# Autodesk Inventor assembly: Whole_Assembly
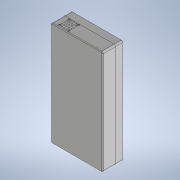
[picture p0: Inventor's stored thumbnail of the model, 180x180]
Saved by Autodesk Inventor 2021 (Build 250183000, 183)
## iProperties
Created: 2020-07-29
Part Number: Whole_Assembly
Document SubType Name: Assembly
Designer: ridvansong
Author: ridvansong
## Documents named in this file (21)
- \\Mac\Home\Documents\OP-1 Project\ipt_files\Whole_Assembly.iam
- \\Mac\Home\Documents\OP-1 Project\ipt_files\Backboard.ipt
- \\Mac\Home\Documents\OP-1 Project\ipt_files\Base.ipt
- \\Mac\Home\Documents\OP-1 Project\ipt_files\Cover.ipt
- \\Mac\Home\Documents\OP-1 Project\ipt_files\RaspPi_Model.ipt
- \\Mac\Home\Documents\OP-1 Project\ipt_files\Fan_Model.ipt
- \\Mac\Home\Documents\OP-1 Project\ipt_files\Battery.ipt
- \\Mac\Home\Documents\OP-1 Project\ipt_files\Battery_Fastener.ipt
- \\Mac\Home\Documents\OP-1 Project\ipt_files\Rotary_Encoder_Model.ipt
- \\Mac\Home\Documents\OP-1 Project\ipt_files\Knob_Base.ipt
- \\Mac\Home\Documents\OP-1 Project\ipt_files\knob.ipt
- \\Mac\Home\Documents\OP-1 Project\ipt_files\Keyboard_Base.ipt
- \\Mac\Home\Documents\OP-1 Project\ipt_files\Small_Button_Base.ipt
- \\Mac\Home\Documents\OP-1 Project\ipt_files\Black_Keyboard_Button_Base.ipt
- \\Mac\Home\Documents\OP-1 Project\ipt_files\Button Prong.ipt
- \\Mac\Home\Documents\OP-1 Project\ipt_files\Black_Keyboard_Button_Prong.ipt
- \\Mac\Home\Documents\OP-1 Project\ipt_files\Keyboard_Prong.ipt
- \\Mac\Home\Documents\OP-1 Project\ipt_files\Small_Button.ipt
- \\Mac\Home\Documents\OP-1 Project\ipt_files\Keyboard Button.ipt
- \\Mac\Home\Documents\OP-1 Project\ipt_files\Black_Keyboard_Button.ipt
- \\Mac\Home\Documents\OP-1 Project\ipt_files\Screen_Model.ipt
## Components (180 placed, 20 different names)
1. Backboard:1 — Mate:1, Mate:3, Mate:4, Mate:15, Mate:16, Mate:17, Mate:18, Angle:1, Angle:2, Angle:3, Angle:4, Mate:25, Mate:35, Mate:37
2. Base:1 — Mate:1, Flush:1, Flush:2, Mate:2, Mate:3, Mate:4, Mate:5, Mate:6, Mate:7, Mate:8, Mate:9, Mate:10, Mate:11, Mate:12, Mate:13, Tangent:1, Tangent:2, Flush:4, Flush:5, Flush:6, Flush:7
3. Cover:1 — Flush:1, Flush:2, Mate:2, Mate:19, Mate:20, Mate:34, Flush:139
4. RaspPi_Model:1 — Mate:8, Mate:9, Mate:10
5. Fan_Model:1 — Mate:5, Mate:6, Mate:7
6. Fan_Model:2 — Mate:11, Mate:12, Mate:13
7. Battery:1 — Tangent:1, Tangent:2, Flush:3
8. Battery_Fastener:1 — Flush:5, Flush:6, Flush:7
9. Rotary_Encoder_Model:1 — Mate:18, Mate:21, Angle:4, Mate:32
10. Rotary_Encoder_Model:2 — Mate:17, Mate:22, Angle:3, Mate:30
11. Rotary_Encoder_Model:3 — Mate:16, Mate:23, Angle:2, Mate:28
12. Rotary_Encoder_Model:4 — Mate:15, Mate:24, Angle:1, Mate:26
13. Knob_Base:1 — Mate:19, Mate:20, Mate:21, Mate:22, Mate:23, Mate:24, Mate:25, Mate:27, Mate:29, Mate:31, Mate:33, Mate:53
14. knob:1 — Mate:26, Mate:27
15. knob:2 — Mate:28, Mate:29
16. knob:3 — Mate:30, Mate:31
17. knob:4 — Mate:32, Mate:33
18. Small_Button_Base:67 — Flush:48, Mate:54, Mate:55, Flush:50, Flush:62, Flush:63, Mate:68, Flush:132, Flush:134
19. Small_Button_Base:68 — Flush:49, Flush:50, Mate:56, Flush:74, Flush:75, Mate:69, Flush:136, Flush:138
20. Black_Keyboard_Button_Base:1 — Flush:53, Flush:54, Flush:55, Flush:56, Flush:57, Mate:64, Mate:65, Flush:107, Flush:108
21. Black_Keyboard_Button_Base:2 — Flush:56, Flush:57, Flush:58, Flush:59, Flush:60, Flush:120, Flush:121
22. Black_Keyboard_Button_Base:3 — Flush:59, Flush:60, Flush:61, Flush:110, Flush:111
23. Black_Keyboard_Button_Base:4 — Flush:62, Flush:63, Flush:64, Flush:65, Flush:66, Mate:66, Flush:123, Flush:124
24. Black_Keyboard_Button_Base:5 — Flush:65, Flush:66, Flush:67, Flush:68, Flush:69, Flush:114, Flush:115
25. Black_Keyboard_Button_Base:6 — Flush:68, Flush:69, Flush:70, Flush:71, Flush:126, Flush:127
26. Black_Keyboard_Button_Base:7 — Flush:71, Flush:72, Flush:74, Flush:117, Flush:118
27. Black_Keyboard_Button_Base:8 — Flush:73, Flush:75, Flush:76, Mate:67, Flush:129, Flush:130
28. Black_Keyboard_Button_Prong:3 — Flush:85, Flush:86, Mate:67
29. Button Prong:31 — Flush:87, Flush:88, Mate:68
30. Button Prong:32 — Flush:89, Flush:90, Mate:69
31. Black_Keyboard_Button:1 — Flush:106, Flush:107, Flush:108, Flush:119
32. Black_Keyboard_Button:2 — Flush:112, Flush:117, Flush:118
33. Black_Keyboard_Button:3 — Flush:109, Flush:110, Flush:111, Flush:122, Flush:131, Flush:133
34. Black_Keyboard_Button:4 — Flush:114, Flush:115, Flush:116
35. Black_Keyboard_Button:5 — Flush:119, Flush:120, Flush:121, Mate:75
36. Black_Keyboard_Button:6 — Flush:122, Flush:123, Flush:124
37. Black_Keyboard_Button:7 — Flush:125, Flush:126, Flush:127
38. Black_Keyboard_Button:8 — Flush:128, Flush:129, Flush:130, Flush:135
39. Small_Button:31 — Flush:131, Flush:135, Flush:136, Flush:138
40. Small_Button:33 — Flush:132, Flush:133, Flush:134
41. Screen_Model:1 — Flush:139, Mate:74, Mate:75
42. Small_Button_Base:16 — Mate:52, Flush:46, Flush:47, Mate:54, Flush:51, Flush:52, Mate:61, Mate:62, Flush:98, Flush:99
43. Small_Button_Base:15 — Mate:52, Flush:46, Flush:47, Mate:53, Mate:63, Flush:101, Flush:102
44. Small_Button_Base:41
45. Small_Button_Base:42
46. Small_Button_Base:43
47. Small_Button_Base:44
48. Small_Button_Base:45
49. Small_Button_Base:46
50. Small_Button_Base:47
51. Small_Button_Base:48
52. Small_Button_Base:49 — Flush:49
53. Small_Button_Base:50
54. Small_Button_Base:51 — Flush:137
55. Small_Button_Base:52
56. Small_Button_Base:53
57. Small_Button_Base:54
58. Keyboard_Base:1 — Mate:34, Mate:35, Mate:37, Flush:34, Flush:35, Mate:50, Flush:54, Mate:70
59. Keyboard_Base:2
60. Keyboard_Base:3 — Flush:58
61. Keyboard_Base:4 — Flush:61
62. Keyboard_Base:5
63. Keyboard_Base:6 — Flush:48, Mate:55
64. Keyboard_Base:7 — Flush:51, Flush:52, Flush:64
65. Keyboard_Base:8 — Flush:67
66. Keyboard_Base:9
67. Keyboard_Base:10 — Flush:70
68. Keyboard_Base:11 — Flush:72
69. Keyboard_Base:12
70. Keyboard_Base:13 — Mate:56, Flush:73
71. Keyboard_Base:14 — Flush:76, Flush:104, Flush:105
72. Small_Button_Base:2 — Flush:34, Flush:35, Flush:36, Flush:37, Mate:50, Mate:51, Mate:60
73. Small_Button_Base:1 — Flush:36, Flush:37, Mate:51, Mate:57, Mate:58, Mate:59
74. Small_Button_Base:55
75. Small_Button_Base:56
76. Small_Button_Base:57 — Flush:53, Flush:55
77. Small_Button_Base:58
78. Small_Button_Base:59
79. Small_Button_Base:60
80. Small_Button_Base:61
81. Small_Button_Base:62
82. Small_Button_Base:63
83. Small_Button_Base:64
84. Small_Button_Base:65 — Flush:95, Flush:97
85. Small_Button_Base:66 — Flush:93, Flush:94
86. Button Prong:2 — Flush:77, Mate:60, Flush:78, Flush:91, Flush:92
87. Button Prong:1 — Mate:57, Mate:58, Mate:59, Flush:77, Flush:78
88. Button Prong:3
89. Button Prong:4
90. Button Prong:5
91. Button Prong:6
92. Button Prong:7 — Flush:82
93. Button Prong:8
94. Button Prong:9
95. Button Prong:10
96. Button Prong:11 — Flush:79
97. Button Prong:12
98. Button Prong:13
99. Button Prong:14 — Mate:71
100. Button Prong:15 — Flush:79, Mate:61, Mate:62, Flush:80, Flush:81, Mate:72
101. Button Prong:16 — Flush:80, Flush:81, Mate:63
102. Button Prong:17
103. Button Prong:18
104. Button Prong:19
105. Button Prong:20
106. Button Prong:21
107. Button Prong:22
108. Button Prong:23
109. Button Prong:24
110. Button Prong:25
111. Button Prong:26
112. Button Prong:27
113. Button Prong:28
114. Button Prong:29
115. Button Prong:30
116. Black_Keyboard_Button_Prong:1 — Mate:64, Flush:82, Mate:65
117. Black_Keyboard_Button_Prong:4
118. Black_Keyboard_Button_Prong:5 — Flush:83, Flush:84, Flush:87, Flush:88
119. Black_Keyboard_Button_Prong:2 — Flush:83, Flush:84, Mate:66
120. Black_Keyboard_Button_Prong:6
121. Black_Keyboard_Button_Prong:7
122. Black_Keyboard_Button_Prong:8 — Flush:85, Flush:86, Flush:89, Flush:90
123. Keyboard_Prong:1 — Flush:91, Flush:92, Mate:70
124. Keyboard_Prong:2
125. Keyboard_Prong:3
126. Keyboard_Prong:4
127. Keyboard_Prong:5
128. Keyboard_Prong:6
129. Keyboard_Prong:7
130. Keyboard_Prong:8
131. Keyboard_Prong:9
132. Keyboard_Prong:10
133. Keyboard_Prong:11
134. Keyboard_Prong:12
135. Keyboard_Prong:13
136. Keyboard_Prong:14
137. Small_Button:1 — Mate:71, Flush:93, Flush:94, Flush:96
138. Small_Button:2 — Flush:95, Flush:96, Flush:97
139. Small_Button:3
140. Small_Button:4
141. Small_Button:5
142. Small_Button:6
143. Small_Button:7
144. Small_Button:8
145. Small_Button:9
146. Small_Button:10
147. Small_Button:11
148. Small_Button:12
149. Small_Button:13
150. Small_Button:14
151. Small_Button:15 — Mate:72, Flush:98, Flush:99, Flush:100, Mate:74
152. Small_Button:16 — Flush:100, Flush:101, Flush:102
153. Small_Button:17
154. Small_Button:18
155. Small_Button:19
156. Small_Button:20
157. Small_Button:21
158. Small_Button:22
159. Small_Button:23
160. Small_Button:24
161. Small_Button:25
162. Small_Button:26
163. Small_Button:27 — Flush:137
164. Small_Button:28
165. Small_Button:29 — Flush:103
166. Small_Button:30
167. Keyboard Button:1 — Flush:103, Flush:104, Flush:105, Flush:128
168. Keyboard Button:2
169. Keyboard Button:3
170. Keyboard Button:4
171. Keyboard Button:5 — Flush:125
172. Keyboard Button:6
173. Keyboard Button:7 — Flush:112, Flush:116
174. Keyboard Button:8
175. Keyboard Button:9
176. Keyboard Button:10
177. Keyboard Button:11 — Flush:109
178. Keyboard Button:12
179. Keyboard Button:13 — Flush:106
180. Keyboard Button:14
## Component patterns: (8 elements, first: Small_Button_Base:16 + Small_Button_Base:15), (14 elements, first: Keyboard_Base:1), (7 elements, first: Small_Button_Base:2 + Small_Button_Base:1), (7 elements, first: Button Prong:2 + Button Prong:1), (8 elements, first: Button Prong:15 + Button Prong:16), (3 elements, first: Black_Keyboard_Button_Prong:1), (4 elements, first: Black_Keyboard_Button_Prong:2), (14 elements, first: Keyboard_Prong:1), (7 elements, first: Small_Button:1 + Small_Button:2), (8 elements, first: Small_Button:15 + Small_Button:16), (14 elements, first: Keyboard Button:1)
## Relationships (171: Flush 104, Mate 61, Angle 4, Tangent 2)
- Mate:1: Backboard:1 ↔ Base:1
- Flush:1: Base:1 ↔ Cover:1
- Flush:2: Base:1 ↔ Cover:1
- Mate:2: Base:1 ↔ Cover:1
- Mate:3 (3 mm): Backboard:1 ↔ Base:1
- Mate:4 (3 mm): Backboard:1 ↔ Base:1
- Mate:5: Base:1 ↔ Fan_Model:1
- Mate:6: Base:1 ↔ Fan_Model:1
- Mate:7: Base:1 ↔ Fan_Model:1
- Mate:8: Base:1 ↔ RaspPi_Model:1
- Mate:9: Base:1 ↔ RaspPi_Model:1
- Mate:10: Base:1 ↔ RaspPi_Model:1
- Mate:11: Base:1 ↔ Fan_Model:2
- Mate:12: Base:1 ↔ Fan_Model:2
- Mate:13: Base:1 ↔ Fan_Model:2
- Tangent:1: Base:1 ↔ Battery:1
- Tangent:2 (15 mm): Base:1 ↔ Battery:1
- Flush:3 (-47.5 mm): Battery:1
- Flush:4 (-134 mm): Base:1
- Mate:14
- Flush:5: Base:1 ↔ Battery_Fastener:1
- Flush:6: Base:1 ↔ Battery_Fastener:1
- Mate:15: Backboard:1 ↔ Rotary_Encoder_Model:4
- Mate:16: Backboard:1 ↔ Rotary_Encoder_Model:3
- Mate:17: Backboard:1 ↔ Rotary_Encoder_Model:2
- Mate:18: Backboard:1 ↔ Rotary_Encoder_Model:1
- Mate:19 (1 mm): Cover:1 ↔ Knob_Base:1
- Mate:20 (1 mm): Cover:1 ↔ Knob_Base:1
- Mate:21: Rotary_Encoder_Model:1 ↔ Knob_Base:1
- Mate:22: Rotary_Encoder_Model:2 ↔ Knob_Base:1
- Mate:23: Rotary_Encoder_Model:3 ↔ Knob_Base:1
- Mate:24: Rotary_Encoder_Model:4 ↔ Knob_Base:1
- Angle:1 (0 deg): Backboard:1 ↔ Rotary_Encoder_Model:4
- Angle:2 (0 deg): Backboard:1 ↔ Rotary_Encoder_Model:3
- Angle:3 (0 deg): Backboard:1 ↔ Rotary_Encoder_Model:2
- Angle:4 (0 deg): Backboard:1 ↔ Rotary_Encoder_Model:1
- Mate:25: Backboard:1 ↔ Knob_Base:1
- Flush:7: Base:1 ↔ Battery_Fastener:1
- Mate:26: Rotary_Encoder_Model:4 ↔ knob:1
- Mate:27: Knob_Base:1 ↔ knob:1
- Mate:28: Rotary_Encoder_Model:3 ↔ knob:2
- Mate:29: Knob_Base:1 ↔ knob:2
- Mate:30: Rotary_Encoder_Model:2 ↔ knob:3
- Mate:31: Knob_Base:1 ↔ knob:3
- Mate:32: Rotary_Encoder_Model:1 ↔ knob:4
- Mate:33: Knob_Base:1 ↔ knob:4
- Mate:34 (1 mm): Cover:1 ↔ Keyboard_Base:1
- Mate:35 (0.25 mm): Backboard:1 ↔ Keyboard_Base:1
- Mate:37: Backboard:1 ↔ Keyboard_Base:1
- Flush:34: Keyboard_Base:1 ↔ Small_Button_Base:2
- Flush:35: Keyboard_Base:1 ↔ Small_Button_Base:2
- Flush:36: Small_Button_Base:2 ↔ Small_Button_Base:1
- Flush:37: Small_Button_Base:2 ↔ Small_Button_Base:1
- Mate:50 (1 mm): Keyboard_Base:1 ↔ Small_Button_Base:2
- Mate:51 (1 mm): Small_Button_Base:2 ↔ Small_Button_Base:1
- Mate:52 (1 mm): Small_Button_Base:16 ↔ Small_Button_Base:15
- Flush:46: Small_Button_Base:16 ↔ Small_Button_Base:15
- Flush:47: Small_Button_Base:16 ↔ Small_Button_Base:15
- Mate:53 (1 mm): Knob_Base:1 ↔ Small_Button_Base:15
- Flush:48: Small_Button_Base:67 ↔ Keyboard_Base:6
- Mate:54 (1 mm): Small_Button_Base:67 ↔ Small_Button_Base:16
- Mate:55 (-6.5 mm): Small_Button_Base:67 ↔ Keyboard_Base:6
- Flush:49: Small_Button_Base:68 ↔ Small_Button_Base:49
- Flush:50: Small_Button_Base:67 ↔ Small_Button_Base:68
- Flush:51: Small_Button_Base:16 ↔ Keyboard_Base:7
- Flush:52: Small_Button_Base:16 ↔ Keyboard_Base:7
- Mate:56 (-6.5 mm): Small_Button_Base:68 ↔ Keyboard_Base:13
- Flush:53: Black_Keyboard_Button_Base:1 ↔ Small_Button_Base:57
- Flush:54: Black_Keyboard_Button_Base:1 ↔ Keyboard_Base:1
- Flush:55: Black_Keyboard_Button_Base:1 ↔ Small_Button_Base:57
- Flush:56: Black_Keyboard_Button_Base:1 ↔ Black_Keyboard_Button_Base:2
- Flush:57: Black_Keyboard_Button_Base:1 ↔ Black_Keyboard_Button_Base:2
- Flush:58: Black_Keyboard_Button_Base:2 ↔ Keyboard_Base:3
- Flush:59: Black_Keyboard_Button_Base:2 ↔ Black_Keyboard_Button_Base:3
- Flush:60: Black_Keyboard_Button_Base:2 ↔ Black_Keyboard_Button_Base:3
- Flush:61: Black_Keyboard_Button_Base:3 ↔ Keyboard_Base:4
- Flush:62: Small_Button_Base:67 ↔ Black_Keyboard_Button_Base:4
- Flush:63: Small_Button_Base:67 ↔ Black_Keyboard_Button_Base:4
- Flush:64: Black_Keyboard_Button_Base:4 ↔ Keyboard_Base:7
- Flush:65: Black_Keyboard_Button_Base:4 ↔ Black_Keyboard_Button_Base:5
- Flush:66: Black_Keyboard_Button_Base:4 ↔ Black_Keyboard_Button_Base:5
- Flush:67: Black_Keyboard_Button_Base:5 ↔ Keyboard_Base:8
- Flush:68: Black_Keyboard_Button_Base:5 ↔ Black_Keyboard_Button_Base:6
- Flush:69: Black_Keyboard_Button_Base:5 ↔ Black_Keyboard_Button_Base:6
- Flush:70: Black_Keyboard_Button_Base:6 ↔ Keyboard_Base:10
- Flush:71: Black_Keyboard_Button_Base:6 ↔ Black_Keyboard_Button_Base:7
- Flush:72: Black_Keyboard_Button_Base:7 ↔ Keyboard_Base:11
- Flush:73: Black_Keyboard_Button_Base:8 ↔ Keyboard_Base:13
- Flush:74: Small_Button_Base:68 ↔ Black_Keyboard_Button_Base:7
- Flush:75: Small_Button_Base:68 ↔ Black_Keyboard_Button_Base:8
- Flush:76: Black_Keyboard_Button_Base:8 ↔ Keyboard_Base:14
- Mate:57 (0.25 mm): Small_Button_Base:1 ↔ Button Prong:1
- Mate:58 (0.25 mm): Small_Button_Base:1 ↔ Button Prong:1
- Mate:59: Small_Button_Base:1 ↔ Button Prong:1
- Flush:77: Button Prong:2 ↔ Button Prong:1
- Mate:60 (0.25 mm): Small_Button_Base:2 ↔ Button Prong:2
- Flush:78: Button Prong:2 ↔ Button Prong:1
- Flush:79: Button Prong:11 ↔ Button Prong:15
- Mate:61 (0.25 mm): Small_Button_Base:16 ↔ Button Prong:15
- Mate:62 (0.25 mm): Small_Button_Base:16 ↔ Button Prong:15
- Flush:80: Button Prong:15 ↔ Button Prong:16
- Flush:81: Button Prong:15 ↔ Button Prong:16
- Mate:63 (0.25 mm): Small_Button_Base:15 ↔ Button Prong:16
- Mate:64 (0.25 mm): Black_Keyboard_Button_Base:1 ↔ Black_Keyboard_Button_Prong:1
- Flush:82: Button Prong:7 ↔ Black_Keyboard_Button_Prong:1
- Mate:65 (0.25 mm): Black_Keyboard_Button_Base:1 ↔ Black_Keyboard_Button_Prong:1
- Flush:83: Black_Keyboard_Button_Prong:5 ↔ Black_Keyboard_Button_Prong:2
- Flush:84: Black_Keyboard_Button_Prong:5 ↔ Black_Keyboard_Button_Prong:2
- Mate:66 (0.25 mm): Black_Keyboard_Button_Base:4 ↔ Black_Keyboard_Button_Prong:2
- Flush:85: Black_Keyboard_Button_Prong:3 ↔ Black_Keyboard_Button_Prong:8
- Flush:86: Black_Keyboard_Button_Prong:3 ↔ Black_Keyboard_Button_Prong:8
- Mate:67 (0.25 mm): Black_Keyboard_Button_Base:8 ↔ Black_Keyboard_Button_Prong:3
- Flush:87: Button Prong:31 ↔ Black_Keyboard_Button_Prong:5
- Flush:88: Button Prong:31 ↔ Black_Keyboard_Button_Prong:5
- Mate:68 (0.25 mm): Small_Button_Base:67 ↔ Button Prong:31
- Flush:89: Button Prong:32 ↔ Black_Keyboard_Button_Prong:8
- Flush:90: Button Prong:32 ↔ Black_Keyboard_Button_Prong:8
- Mate:69 (0.25 mm): Small_Button_Base:68 ↔ Button Prong:32
- Flush:91: Button Prong:2 ↔ Keyboard_Prong:1
- Flush:92: Button Prong:2 ↔ Keyboard_Prong:1
- Mate:70 (0.25 mm): Keyboard_Base:1 ↔ Keyboard_Prong:1
- Mate:71: Button Prong:14 ↔ Small_Button:1
- Flush:93: Small_Button_Base:66 ↔ Small_Button:1
- Flush:94: Small_Button_Base:66 ↔ Small_Button:1
- Flush:95: Small_Button_Base:65 ↔ Small_Button:2
- Flush:96: Small_Button:1 ↔ Small_Button:2
- Flush:97: Small_Button_Base:65 ↔ Small_Button:2
- Mate:72: Button Prong:15 ↔ Small_Button:15
- Flush:98: Small_Button_Base:16 ↔ Small_Button:15
- Flush:99: Small_Button_Base:16 ↔ Small_Button:15
- Flush:100: Small_Button:15 ↔ Small_Button:16
- Flush:101: Small_Button_Base:15 ↔ Small_Button:16
- Flush:102: Small_Button_Base:15 ↔ Small_Button:16
- Flush:103: Small_Button:29 ↔ Keyboard Button:1
- Flush:104: Keyboard_Base:14 ↔ Keyboard Button:1
- Flush:105: Keyboard_Base:14 ↔ Keyboard Button:1
- Flush:106: Black_Keyboard_Button:1 ↔ Keyboard Button:13
- Flush:107: Black_Keyboard_Button_Base:1 ↔ Black_Keyboard_Button:1
- Flush:108: Black_Keyboard_Button_Base:1 ↔ Black_Keyboard_Button:1
- Flush:109: Black_Keyboard_Button:3 ↔ Keyboard Button:11
- Flush:110: Black_Keyboard_Button_Base:3 ↔ Black_Keyboard_Button:3
- Flush:111: Black_Keyboard_Button_Base:3 ↔ Black_Keyboard_Button:3
- Flush:112: Black_Keyboard_Button:2 ↔ Keyboard Button:7
- Flush:114: Black_Keyboard_Button_Base:5 ↔ Black_Keyboard_Button:4
- Flush:115: Black_Keyboard_Button_Base:5 ↔ Black_Keyboard_Button:4
- Flush:116: Black_Keyboard_Button:4 ↔ Keyboard Button:7
- Flush:117: Black_Keyboard_Button_Base:7 ↔ Black_Keyboard_Button:2
- Flush:118: Black_Keyboard_Button_Base:7 ↔ Black_Keyboard_Button:2
- Flush:119: Black_Keyboard_Button:1 ↔ Black_Keyboard_Button:5
- Flush:120: Black_Keyboard_Button_Base:2 ↔ Black_Keyboard_Button:5
- Flush:121: Black_Keyboard_Button_Base:2 ↔ Black_Keyboard_Button:5
- Flush:122: Black_Keyboard_Button:3 ↔ Black_Keyboard_Button:6
- Flush:123: Black_Keyboard_Button_Base:4 ↔ Black_Keyboard_Button:6
- Flush:124: Black_Keyboard_Button_Base:4 ↔ Black_Keyboard_Button:6
- Flush:125: Black_Keyboard_Button:7 ↔ Keyboard Button:5
- Flush:126: Black_Keyboard_Button_Base:6 ↔ Black_Keyboard_Button:7
- Flush:127: Black_Keyboard_Button_Base:6 ↔ Black_Keyboard_Button:7
- Flush:128: Black_Keyboard_Button:8 ↔ Keyboard Button:1
- Flush:129: Black_Keyboard_Button_Base:8 ↔ Black_Keyboard_Button:8
- Flush:130: Black_Keyboard_Button_Base:8 ↔ Black_Keyboard_Button:8
- Flush:131: Black_Keyboard_Button:3 ↔ Small_Button:31
- Flush:132: Small_Button_Base:67 ↔ Small_Button:33
- Flush:133: Black_Keyboard_Button:3 ↔ Small_Button:33
- Flush:134: Small_Button_Base:67 ↔ Small_Button:33
- Flush:135: Black_Keyboard_Button:8 ↔ Small_Button:31
- Flush:136: Small_Button_Base:68 ↔ Small_Button:31
- Flush:137: Small_Button_Base:51 ↔ Small_Button:27
- Flush:138: Small_Button_Base:68 ↔ Small_Button:31
- Flush:139 (1 mm): Cover:1 ↔ Screen_Model:1
- Mate:74 (2.5 mm): Screen_Model:1 ↔ Small_Button:15
- Mate:75 (2.5 mm): Black_Keyboard_Button:5 ↔ Screen_Model:1
